# Autodesk Inventor assembly: DoublePulley
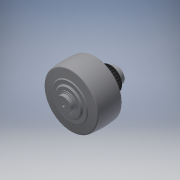
[picture p0: Inventor's stored thumbnail of the model, 180x180]
Saved by Autodesk Inventor 2016 (Build 200138000, 138)
## iProperties
Created: 2017-01-15
Part Number: DoublePulley
Document SubType Name: Assembly
Designer: Kyle
Author: Kyle
## Documents named in this file (7)
- F:\FRC\2017\DriveTrainRev3\Individual Parts\DoublePulley.iam
- F:\FRC\2017\DriveTrainRev3\Individual Parts\.5Bearing.ipt
- F:\FRC\2017\DriveTrainRev3\Individual Parts\4x2Colson.ipt
- F:\FRC\2017\DriveTrainRev3\Individual Parts\24t9MMPulley6mm.ipt
- F:\FRC\2017\DriveTrainRev3\Individual Parts\24t9MMPulleyExtension.ipt
- F:\FRC\2017\DriveTrainRev3\Individual Parts\.106Spacer.ipt
- F:\FRC\2017\DriveTrainRev3\Individual Parts\.5HexShaft3.875in.ipt
## Components (8 placed, 6 different names)
1. .5Bearing:1 — Mate:3, Mate:16, Flush:1
2. 4x2Colson:1 — Mate:3, Mate:11
3. 24t9MMPulley6mm:1 — Mate:4, Mate:5, Mate:6, Mate:7, Mate:11
4. 24t9MMPulley6mm:2 — Mate:7, Mate:8, Mate:9, Mate:13
5. 24t9MMPulleyExtension:1 — Mate:4, Mate:5, Mate:6, Mate:8, Mate:9
6. .106Spacer:1 — Mate:13, Mate:15
7. .5Bearing:2 — Mate:15
8. .5HexShaft3.875in:1 — Mate:16, Flush:1
## Relationships (12: Mate 11, Flush 1)
- Mate:3: .5Bearing:1 ↔ 4x2Colson:1
- Mate:4: 24t9MMPulley6mm:1 ↔ 24t9MMPulleyExtension:1
- Mate:5: 24t9MMPulley6mm:1 ↔ 24t9MMPulleyExtension:1
- Mate:6: 24t9MMPulley6mm:1 ↔ 24t9MMPulleyExtension:1
- Mate:7: 24t9MMPulley6mm:1 ↔ 24t9MMPulley6mm:2
- Mate:8: 24t9MMPulley6mm:2 ↔ 24t9MMPulleyExtension:1
- Mate:9: 24t9MMPulley6mm:2 ↔ 24t9MMPulleyExtension:1
- Mate:11: 4x2Colson:1 ↔ 24t9MMPulley6mm:1
- Mate:13: 24t9MMPulley6mm:2 ↔ .106Spacer:1
- Mate:15: .106Spacer:1 ↔ .5Bearing:2
- Mate:16: .5Bearing:1 ↔ .5HexShaft3.875in:1
- Flush:1: .5Bearing:1 ↔ .5HexShaft3.875in:1
